# Autodesk Inventor assembly: base_body_remake
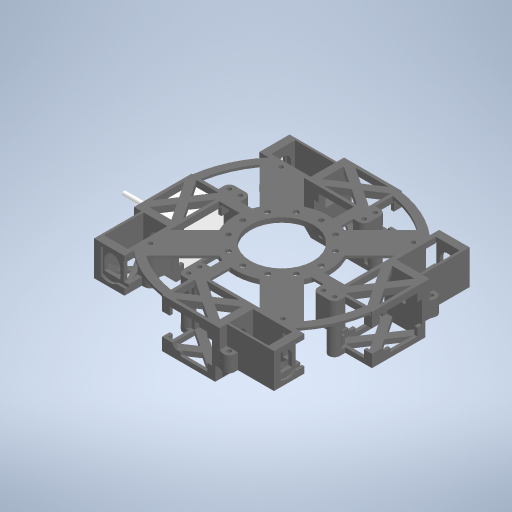
[picture p0: Inventor's stored thumbnail of the model, 512x512]
Saved by Autodesk Inventor 2024.1 (Build 281209000, 209)
## iProperties
Created: 2024-07-05
Part Number: base_body_remake
Document SubType Name: Assembly
Designer: hibik
Author: hibik
## Documents named in this file (4)
- C:\Users\hibik\Desktop\ロボメカ\Rescue\2年\子機_本選\base_body_remake.iam
- C:\Users\hibik\Desktop\ロボメカ\Rescue\2年\子機_本選\body_upper_remake.ipt
- C:\Users\hibik\Desktop\ロボメカ\Rescue\2年\子機_本選\body_under_remake.ipt
- C:\Users\hibik\Desktop\ロボメカ\Rescue\2年\子機_本選\Motor.ipt
## Components (6 placed, 3 different names)
1. body_upper_remake:1 — メイト:2, メイト:3, メイト:4, 挿入:1, メイト:5, 挿入:2, 挿入:3, 挿入:4, メイト:6, メイト:7, メイト:8
2. Motor:1 — メイト:2, メイト:3, メイト:4
3. body_under_remake:1 — 挿入:1, メイト:5
4. body_under_remake:2 — 挿入:2, メイト:6
5. body_under_remake:3 — 挿入:4, メイト:8
6. body_under_remake:4 — 挿入:3, メイト:7
## Relationships (11: Mate 7, Insert 4)
- メイト:2 [Mate]: body_upper_remake:1 ↔ Motor:1
- メイト:3 [Mate]: body_upper_remake:1 ↔ Motor:1
- メイト:4 [Mate]: body_upper_remake:1 ↔ Motor:1
- 挿入:1 [Insert]: body_upper_remake:1 ↔ body_under_remake:1
- メイト:5 [Mate]: body_upper_remake:1 ↔ body_under_remake:1
- 挿入:2 [Insert]: body_upper_remake:1 ↔ body_under_remake:2
- 挿入:3 [Insert]: body_upper_remake:1 ↔ body_under_remake:4
- 挿入:4 [Insert]: body_upper_remake:1 ↔ body_under_remake:3
- メイト:6 [Mate]: body_upper_remake:1 ↔ body_under_remake:2
- メイト:7 [Mate]: body_upper_remake:1 ↔ body_under_remake:4
- メイト:8 [Mate]: body_upper_remake:1 ↔ body_under_remake:3
